# Autodesk Inventor assembly: main
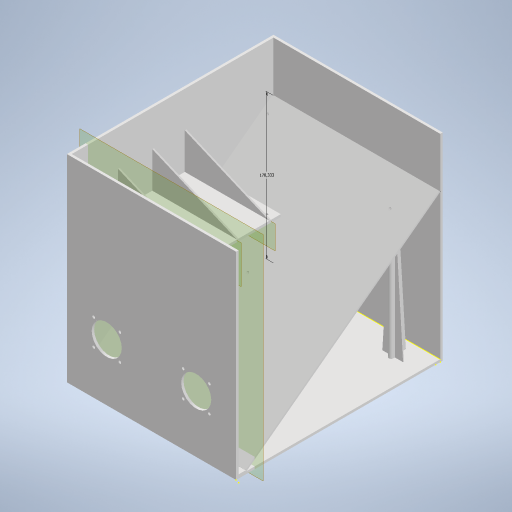
[picture p0: Inventor's stored thumbnail of the model, 512x512]
Saved by Autodesk Inventor 2024 (Build 280153000, 153)
## iProperties
Created: 2026-03-22
Part Number: main
Document SubType Name: Assembly
Designer: schar
Author: schar
## Documents named in this file (3)
- C:\Users\schar\Desktop\tenSwitcHP\models\main.iam
- C:\Users\schar\Desktop\tenSwitcHP\models\rack.ipt
- C:\Users\schar\Desktop\tenSwitcHP\models\base_main_pcb.ipt
## Components (2 placed, 2 different names)
1. rack:1 — Mate:1, Flush:1, Mate:2
2. base_main_pcb:1 — Mate:1, Flush:1, Mate:2
## Relationships (3: Mate 2, Flush 1)
- Mate:1: rack:1 ↔ base_main_pcb:1
- Flush:1: rack:1 ↔ base_main_pcb:1
- Mate:2: rack:1 ↔ base_main_pcb:1
